# Autodesk Inventor assembly: Gamepad_Right
Saved by Autodesk Inventor 2014 SP1 (Build 180222100, 222)
## iProperties
Created: 2014-02-22
Part Number: Gamepad_Right
Document SubType Name: Assembly
Designer: tuleu
Author: tuleu
## Documents named in this file (5)
- C:\Users\tuleu\Documents\giant-snes-gamepad\cad\Gamepad_Right.iam
- C:\Users\tuleu\Documents\giant-snes-gamepad\cad\Trigger_Cell.iam
- C:\Users\tuleu\Documents\giant-snes-gamepad\cad\Start_Cell.iam
- C:\Users\tuleu\Documents\giant-snes-gamepad\cad\Circle_Cell.iam
- C:\Users\tuleu\Documents\giant-snes-gamepad\cad\Foam_Right.ipt
## Components (7 placed, 4 different names)
1. Trigger_Cell:1 [sub-assembly]
2. Start_Cell:1 [sub-assembly]
3. Circle_Cell:1 [sub-assembly]
4. Circle_Cell:2 [sub-assembly]
5. Circle_Cell:3 [sub-assembly]
6. Circle_Cell:4 [sub-assembly]
7. Foam_Right:1
## Relationships (2: Mate 2)
- [Mate]: Circle_Cell:1 ↔ Circle_Cell:3
- [Mate]: Circle_Cell:2 ↔ Circle_Cell:4
